# Autodesk Inventor assembly: Middleplate Assy
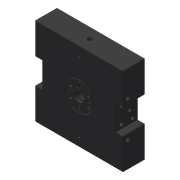
[picture p0: Inventor's stored thumbnail of the model, 180x180]
Saved by Autodesk Inventor 2022 Beta2 (Build 260130000, 130) ContinuousBuild 0
## iProperties
Shininess: 64.0
Length Units: 11269
Angle Units: 11279
Time Units: 11290
Mass Units: 11283
Length Display Precision: 3
Angle Display Precision: 2
Compacted: True
Part Number: Middleplate Assy
Document SubType Name: Assembly
Created: 2003-04-07
Designer: demo
Density: 0.0
Volumn: 0.0
Area: 0.0
PropertySet Name: Model Information
Control State: 0
Master: False
Checked Out: False
Author: demo
## Documents named in this file (4)
- C:\Autodesk Inventor 2021 Intro Practice Files\Mold Assembly\Middleplate Assy.iam
- C:\Autodesk Inventor 2021 Intro Practice Files\Mold Assembly\middleplate.ipt
- C:\Autodesk Inventor 2021 Intro Practice Files\Mold Assembly\Cavity-middle.ipt
- C:\Autodesk Inventor 2021 Intro Practice Files\Mold Assembly\Core.ipt
## Components (3 placed, 3 different names)
1. middleplate:1 — Mate:1, Flush:1, Mate:4
2. Cavity-middle:1 — Mate:1, Flush:1, Mate:3
3. Core:1 — Mate:3, Mate:4
## Relationships (4: Mate 3, Flush 1)
- Mate:1: middleplate:1 ↔ Cavity-middle:1
- Flush:1: middleplate:1 ↔ Cavity-middle:1
- Mate:3: Cavity-middle:1 ↔ Core:1
- Mate:4: middleplate:1 ↔ Core:1
